# Autodesk Inventor assembly: TestMergerWseat
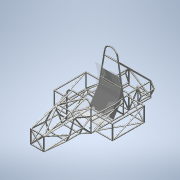
[picture p0: Inventor's stored thumbnail of the model, 180x180]
Saved by Autodesk Inventor 2021 (Build 250183000, 183)
## iProperties
Created: 2020-10-11
Part Number: TestMergerWseat
Document SubType Name: Assembly
Designer: qv17m
_SolveAssemblyDoc: Frame Generator Solve Assembly
_Version: 25.0.0
Author: qv17m
## Documents named in this file (11)
- C:\Users\qv17m\Documents\Inventor\FSAE\FullCarV1.1\FullCarV1.1\FullCarV1.1.iam
- C:\Users\qv17m\Documents\Inventor\FSAE\FullCarV1.1\FullCarV1.1\FSAE_Frame.0007.ipt
- C:\Users\qv17m\Documents\Inventor\FSAE\FullCarV1.1\FullCarV1.1\DesignReviewOct_10 - Copy.ipt
- C:\Users\qv17m\Documents\Inventor\FSAE\FullCarV1.1\FullCarV1.1\Frame\Seat3DSketch.ipt
- C:\Users\qv17m\Documents\Inventor\FSAE\FullCarV1.1\FullCarV1.1\Frame\Seat tab to frame mount.ipt
- C:\Users\qv17m\Documents\Inventor\FSAE\FullCarV1.1\FullCarV1.1\Frame\Seat tabsnew.ipt
- C:\Users\qv17m\Documents\Inventor\FSAE\FullCarV1.1\FullCarV1.1\Frame\harness attachments.ipt
- C:\Users\qv17m\Documents\Inventor\FSAE\FullCarV1.1\FullCarV1.1\FullFrame Oct 13\FullFrameOct13.iam
- C:\Users\qv17m\Documents\Inventor\FSAE\GLVBattery.ipt
- C:\Users\qv17m\Documents\Inventor\FSAE\FullCarV1.1\FullCarV1.1\Firewall\FirewallTrapezoid.ipt
- C:\Users\qv17m\Documents\Inventor\FSAE\FullCarV1.1\FullCarV1.1\Firewall\FirewallDiagonal.ipt
## Components (16 placed, 10 different names)
1. FSAE_Frame.0007:1 — Mate:1
2. DesignReviewOct_10 - Copy:1 — Mate:1
3. FullFrameOct13:1 [sub-assembly] — Mate:57, Mate:58, Mate:59, Mate:60, Angle:1, Mate:61, Mate:62, Mate:63, Mate:64, Mate:65, Mate:66, Mate:67
4. Seat3DSketch:2 — Mate:53, Mate:54, Mate:55
5. Seat tab to frame mount:1 — Mate:41, Mate:42, Mate:63, Mate:67, Mate:68
6. Seat tab to frame mount:2 — Mate:40, Mate:62
7. Seat tab to frame mount:3 — Mate:52, Mate:56, Mate:65, Mate:66, Mate:68
8. Seat tab to frame mount:4 — Mate:38, Mate:39, Mate:64
9. Seat tabsnew:1 — Mate:38, Mate:39, Mate:40, Mate:53, Mate:54, Mate:55
10. Seat tabsnew:2 — Mate:41, Mate:42, Mate:52, Mate:56
11. harness attachments:1 — Mate:61
12. harness attachments:2 — Mate:59, Mate:60, Angle:1
13. harness attachments:3 — Mate:57, Mate:58
14. GLVBattery:1
15. FirewallTrapezoid:1
16. FirewallDiagonal:1
## Relationships (24: Mate 23, Angle 1)
- Mate:1: FSAE_Frame.0007:1 ↔ DesignReviewOct_10 - Copy:1
- Mate:38 (6.35 mm): Seat tab to frame mount:4 ↔ Seat tabsnew:1
- Mate:39: Seat tab to frame mount:4 ↔ Seat tabsnew:1
- Mate:40: Seat tab to frame mount:2 ↔ Seat tabsnew:1
- Mate:41: Seat tab to frame mount:1 ↔ Seat tabsnew:2
- Mate:42: Seat tab to frame mount:1 ↔ Seat tabsnew:2
- Mate:52 (6.35 mm): Seat tab to frame mount:3 ↔ Seat tabsnew:2
- Mate:53: Seat3DSketch:2 ↔ Seat tabsnew:1
- Mate:54: Seat3DSketch:2 ↔ Seat tabsnew:1
- Mate:55 (-6.35 mm): Seat3DSketch:2 ↔ Seat tabsnew:1
- Mate:56: Seat tab to frame mount:3 ↔ Seat tabsnew:2
- Mate:57: FullFrameOct13:1 ↔ harness attachments:3
- Mate:58: FullFrameOct13:1 ↔ harness attachments:3
- Mate:59: FullFrameOct13:1 ↔ harness attachments:2
- Mate:60: FullFrameOct13:1 ↔ harness attachments:2
- Angle:1 (90 deg): FullFrameOct13:1 ↔ harness attachments:2
- Mate:61: FullFrameOct13:1 ↔ harness attachments:1
- Mate:62: FullFrameOct13:1 ↔ Seat tab to frame mount:2
- Mate:63: FullFrameOct13:1 ↔ Seat tab to frame mount:1
- Mate:64: FullFrameOct13:1 ↔ Seat tab to frame mount:4
- Mate:65: FullFrameOct13:1 ↔ Seat tab to frame mount:3
- Mate:66: FullFrameOct13:1 ↔ Seat tab to frame mount:3
- Mate:67: FullFrameOct13:1 ↔ Seat tab to frame mount:1
- Mate:68: Seat tab to frame mount:1 ↔ Seat tab to frame mount:3
